# Autodesk Inventor assembly: Assembly_for_al_2l
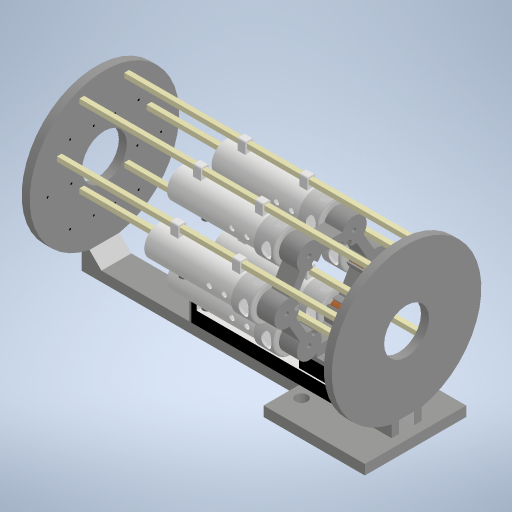
[picture p0: Inventor's stored thumbnail of the model, 512x512]
Saved by Autodesk Inventor 2023 (Build 270158000, 158)
## iProperties
Created: 2022-11-03
Part Number: Assembly_for_al_2l
Document SubType Name: Assembly
Designer: Admin
Author: Admin
## Documents named in this file (10)
- D:\multimate\Mouse_restrainer_V3\Assembly_for_al_2l.iam
- D:\multimate\Mouse_restrainer_V3\base2.ipt
- D:\multimate\Mouse_restrainer_V3\linear trail.ipt
- D:\multimate\Mouse_restrainer_V3\motor on trail.ipt
- D:\multimate\Mouse_restrainer_V3\support_electrical_magnets.ipt
- D:\multimate\Mouse_restrainer_V3\stock.ipt
- D:\multimate\Mouse_restrainer_V3\electromagnet.ipt
- D:\multimate\Mouse_restrainer_V3\restrainer.iam
- D:\multimate\Mouse_restrainer_V3\micro_magnets_2mm1mm.ipt
- D:\multimate\Mouse_restrainer_V3\28 motor NEMA11.ipt
## Components (47 placed, 9 different names)
1. base2:1 — Rigid:1, Rigid:3, Rigid:11, Rigid:12, Rigid:13, Rigid:14, Rigid:15, Rotational:18, Rotational:19, Rotational:20, Rigid:17, Rotational:21, Rotational:22, Rotational:23, Rotational:24, Rotational:25, Rotational:26, Rotational:27, Rotational:28
2. linear trail:1 — Rigid:1, Cylindrical:1, Angle:1, Rigid:18
3. motor on trail:1 — Cylindrical:1, Angle:1, Rigid:2
4. support_electrical_magnets:1 — Rigid:2, Rotational:1, Rotational:2, Rotational:3, Rotational:4, Rotational:5, Rotational:6
5. stock:1 — Slider:2, Rigid:14
6. stock:2 — Slider:3, Rigid:13
7. stock:3 — Rigid:3, Slider:6
8. stock:4 — Slider:1, Rigid:12
9. stock:5 — Slider:5, Rigid:11
10. stock:6 — Slider:4, Rigid:15
11. electromagnet:1 — Rotational:5
12. electromagnet:2 — Rotational:1
13. electromagnet:3 — Rotational:6
14. electromagnet:4 — Rotational:3
15. electromagnet:5 — Rotational:4
16. electromagnet:6 — Rotational:2
17. restrainer:1 [sub-assembly] — Slider:1, Rotational:15, Rotational:16
18. restrainer:2 [sub-assembly] — Slider:6, Rotational:7, Rotational:8
19. restrainer:3 [sub-assembly] — Slider:2, Rotational:13, Rotational:14
20. restrainer:4 [sub-assembly] — Slider:3, Rigid:16, Rotational:17
21. restrainer:5 [sub-assembly] — Slider:4, Rotational:11, Rotational:12
22. restrainer:6 [sub-assembly] — Slider:5, Rotational:9, Rotational:10
23. micro_magnets_2mm1mm:1 — Rotational:7
24. micro_magnets_2mm1mm:2 — Rotational:8
25. micro_magnets_2mm1mm:3 — Rotational:9
26. micro_magnets_2mm1mm:4 — Rotational:10
27. micro_magnets_2mm1mm:5 — Rotational:11
28. micro_magnets_2mm1mm:6 — Rotational:12
29. micro_magnets_2mm1mm:7 — Rotational:13
30. micro_magnets_2mm1mm:8 — Rotational:14
31. micro_magnets_2mm1mm:9 — Rotational:15
32. micro_magnets_2mm1mm:10 — Rigid:16
33. micro_magnets_2mm1mm:11 — Rotational:16
34. micro_magnets_2mm1mm:12 — Rotational:17
35. micro_magnets_2mm1mm:13 — Rotational:18
36. micro_magnets_2mm1mm:14 — Rigid:17
37. micro_magnets_2mm1mm:15 — Rotational:19
38. micro_magnets_2mm1mm:16 — Rotational:21
39. micro_magnets_2mm1mm:17 — Rotational:20
40. micro_magnets_2mm1mm:18 — Rotational:25
41. micro_magnets_2mm1mm:19 — Rotational:22
42. micro_magnets_2mm1mm:20 — Rotational:26
43. micro_magnets_2mm1mm:21 — Rotational:23
44. micro_magnets_2mm1mm:22 — Rotational:27
45. micro_magnets_2mm1mm:23 — Rotational:24
46. micro_magnets_2mm1mm:24 — Rotational:28
47. 28 motor NEMA11:1 — Rigid:18
## Relationships (47: RevoluteJoint 28, WeldJoint 11, TranslationJoint 6, CylindricalJoint 1, Angle 1)
- Rigid:1 [WeldJoint]: base2:1 ↔ linear trail:1
- Cylindrical:1: linear trail:1 ↔ motor on trail:1
- Angle:1 (0 deg): linear trail:1 ↔ motor on trail:1
- Rigid:2 [WeldJoint]: motor on trail:1 ↔ support_electrical_magnets:1
- Rigid:3 [WeldJoint]: base2:1 ↔ stock:3
- Rotational:1 [RevoluteJoint]: support_electrical_magnets:1 ↔ electromagnet:2
- Rotational:2 [RevoluteJoint]: support_electrical_magnets:1 ↔ electromagnet:6
- Rotational:3 [RevoluteJoint]: support_electrical_magnets:1 ↔ electromagnet:4
- Rotational:4 [RevoluteJoint]: support_electrical_magnets:1 ↔ electromagnet:5
- Rotational:5 [RevoluteJoint]: support_electrical_magnets:1 ↔ electromagnet:1
- Rotational:6 [RevoluteJoint]: support_electrical_magnets:1 ↔ electromagnet:3
- Slider:1 [TranslationJoint]: stock:4 ↔ restrainer:1
- Slider:2 [TranslationJoint]: stock:1 ↔ restrainer:3
- Slider:3 [TranslationJoint]: stock:2 ↔ restrainer:4
- Slider:4 [TranslationJoint]: stock:6 ↔ restrainer:5
- Slider:5 [TranslationJoint]: stock:5 ↔ restrainer:6
- Slider:6 [TranslationJoint]: stock:3 ↔ restrainer:2
- Rigid:11 [WeldJoint]: base2:1 ↔ stock:5
- Rigid:12 [WeldJoint]: base2:1 ↔ stock:4
- Rigid:13 [WeldJoint]: base2:1 ↔ stock:2
- Rigid:14 [WeldJoint]: base2:1 ↔ stock:1
- Rigid:15 [WeldJoint]: base2:1 ↔ stock:6
- Rotational:7 [RevoluteJoint]: restrainer:2 ↔ micro_magnets_2mm1mm:1
- Rotational:8 [RevoluteJoint]: restrainer:2 ↔ micro_magnets_2mm1mm:2
- Rotational:9 [RevoluteJoint]: restrainer:6 ↔ micro_magnets_2mm1mm:3
- Rotational:10 [RevoluteJoint]: restrainer:6 ↔ micro_magnets_2mm1mm:4
- Rotational:11 [RevoluteJoint]: restrainer:5 ↔ micro_magnets_2mm1mm:5
- Rotational:12 [RevoluteJoint]: restrainer:5 ↔ micro_magnets_2mm1mm:6
- Rotational:13 [RevoluteJoint]: restrainer:3 ↔ micro_magnets_2mm1mm:7
- Rotational:14 [RevoluteJoint]: restrainer:3 ↔ micro_magnets_2mm1mm:8
- Rotational:15 [RevoluteJoint]: restrainer:1 ↔ micro_magnets_2mm1mm:9
- Rotational:16 [RevoluteJoint]: restrainer:1 ↔ micro_magnets_2mm1mm:11
- Rigid:16 [WeldJoint]: restrainer:4 ↔ micro_magnets_2mm1mm:10
- Rotational:17 [RevoluteJoint]: restrainer:4 ↔ micro_magnets_2mm1mm:12
- Rotational:18 [RevoluteJoint]: base2:1 ↔ micro_magnets_2mm1mm:13
- Rotational:19 [RevoluteJoint]: base2:1 ↔ micro_magnets_2mm1mm:15
- Rotational:20 [RevoluteJoint]: base2:1 ↔ micro_magnets_2mm1mm:17
- Rigid:17 [WeldJoint]: base2:1 ↔ micro_magnets_2mm1mm:14
- Rotational:21 [RevoluteJoint]: base2:1 ↔ micro_magnets_2mm1mm:16
- Rotational:22 [RevoluteJoint]: base2:1 ↔ micro_magnets_2mm1mm:19
- Rotational:23 [RevoluteJoint]: base2:1 ↔ micro_magnets_2mm1mm:21
- Rotational:24 [RevoluteJoint]: base2:1 ↔ micro_magnets_2mm1mm:23
- Rotational:25 [RevoluteJoint]: base2:1 ↔ micro_magnets_2mm1mm:18
- Rotational:26 [RevoluteJoint]: base2:1 ↔ micro_magnets_2mm1mm:20
- Rotational:27 [RevoluteJoint]: base2:1 ↔ micro_magnets_2mm1mm:22
- Rotational:28 [RevoluteJoint]: base2:1 ↔ micro_magnets_2mm1mm:24
- Rigid:18 [WeldJoint]: linear trail:1 ↔ 28 motor NEMA11:1
